# Autodesk Inventor assembly: Final
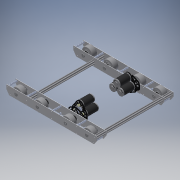
[picture p0: Inventor's stored thumbnail of the model, 180x180]
Saved by Autodesk Inventor 2016 (Build 200138000, 138)
## iProperties
Created: 2017-01-19
Part Number: Final
Document SubType Name: Assembly
Designer: Kyle
Author: Kyle
## Documents named in this file (8)
- C:\Users\Kyle\Documents\FRC1073\FRC1073-CAD\DriveTrain\Final.iam
- C:\Users\Kyle\Documents\FRC1073\FRC1073-CAD\DriveTrain\OutsidePlate.ipt
- C:\Users\Kyle\Documents\FRC1073\FRC1073-CAD\DriveTrain\Individual Parts\Mock 8020 28.25in.ipt
- C:\Users\Kyle\Documents\FRC1073\FRC1073-CAD\DriveTrain\InsidePlate.ipt
- C:\Users\Kyle\Documents\FRC1073\FRC1073-CAD\DriveTrain\Individual Parts\3.625Churro.ipt
- C:\Users\Kyle\Documents\FRC1073\FRC1073-CAD\DriveTrain\Individual Parts\SinglePulley.iam
- C:\Users\Kyle\Documents\FRC1073\FRC1073-CAD\DriveTrain\Individual Parts\DoublePulley.iam
- C:\Users\Kyle\Documents\FRC1073\FRC1073-CAD\DriveTrain\Individual Parts\DoublePulleyGearbox.iam
## Components (32 placed, 7 different names)
1. OutsidePlate:1 — Mate:1, Mate:2, Flush:1, Flush:2, Mate:3, Flush:3, Flush:4, Mate:4, Mate:5, Mate:6, Mate:7, Mate:8, Mate:9, Mate:10, Mate:11, Mate:12, Mate:29, Mate:30, Mate:31, Mate:32, Mate:33, Mate:34, Mate:37, Mate:38
2. Mock 8020 28.25in:1 — Mate:2, Flush:1, Flush:2, Mate:14
3. Mock 8020 28.25in:2 — Mate:1, Mate:3
4. InsidePlate:1 — Flush:3, Flush:4, Mate:13, Mate:42
5. 3.625Churro:1 — Mate:11
6. 3.625Churro:2 — Mate:10, Mate:13
7. 3.625Churro:3 — Mate:12
8. 3.625Churro:4 — Mate:9
9. 3.625Churro:5 — Mate:7
10. 3.625Churro:6 — Mate:8
11. 3.625Churro:7 — Mate:6
12. 3.625Churro:8 — Mate:4
13. 3.625Churro:9 — Mate:5
14. OutsidePlate:2 — Mate:14, Mate:15, Mate:16, Mate:17, Mate:18, Mate:19, Mate:20, Mate:21, Mate:22, Mate:23, Flush:5, Flush:6, Mate:35, Mate:36, Mate:39, Mate:40
15. 3.625Churro:10 — Mate:15
16. 3.625Churro:11 — Mate:16
17. 3.625Churro:12 — Mate:17
18. 3.625Churro:13 — Mate:18
19. 3.625Churro:14 — Mate:19, Mate:24
20. 3.625Churro:15 — Mate:21
21. 3.625Churro:16 — Mate:20
22. 3.625Churro:17 — Mate:23
23. 3.625Churro:18 — Mate:22
24. InsidePlate:2 — Flush:5, Flush:6, Mate:24, Mate:25, Mate:26, Mate:27, Mate:28, Mate:41
25. SinglePulley:1 [sub-assembly] — Mate:31, Mate:32
26. SinglePulley:2 [sub-assembly] — Mate:29, Mate:30
27. SinglePulley:3 [sub-assembly] — Mate:25, Mate:26
28. SinglePulley:4 [sub-assembly] — Mate:27, Mate:28
29. DoublePulley:1 [sub-assembly] — Mate:33, Mate:34
30. DoublePulley:2 [sub-assembly] — Mate:35, Mate:36
31. DoublePulleyGearbox:1 [sub-assembly] — Mate:37, Mate:38, Mate:42
32. DoublePulleyGearbox:2 [sub-assembly] — Mate:39, Mate:40, Mate:41
## Relationships (48: Mate 42, Flush 6)
- Mate:1: OutsidePlate:1 ↔ Mock 8020 28.25in:2
- Mate:2: OutsidePlate:1 ↔ Mock 8020 28.25in:1
- Flush:1 (6.35 mm): OutsidePlate:1 ↔ Mock 8020 28.25in:1
- Flush:2 (6.35 mm): OutsidePlate:1 ↔ Mock 8020 28.25in:1
- Mate:3: OutsidePlate:1 ↔ Mock 8020 28.25in:2
- Flush:3: OutsidePlate:1 ↔ InsidePlate:1
- Flush:4: OutsidePlate:1 ↔ InsidePlate:1
- Mate:4: OutsidePlate:1 ↔ 3.625Churro:8
- Mate:5: OutsidePlate:1 ↔ 3.625Churro:9
- Mate:6: OutsidePlate:1 ↔ 3.625Churro:7
- Mate:7: OutsidePlate:1 ↔ 3.625Churro:5
- Mate:8: OutsidePlate:1 ↔ 3.625Churro:6
- Mate:9: OutsidePlate:1 ↔ 3.625Churro:4
- Mate:10: OutsidePlate:1 ↔ 3.625Churro:2
- Mate:11: OutsidePlate:1 ↔ 3.625Churro:1
- Mate:12: OutsidePlate:1 ↔ 3.625Churro:3
- Mate:13: InsidePlate:1 ↔ 3.625Churro:2
- Mate:14: Mock 8020 28.25in:1 ↔ OutsidePlate:2
- Mate:15: OutsidePlate:2 ↔ 3.625Churro:10
- Mate:16: OutsidePlate:2 ↔ 3.625Churro:11
- Mate:17: OutsidePlate:2 ↔ 3.625Churro:12
- Mate:18: OutsidePlate:2 ↔ 3.625Churro:13
- Mate:19: OutsidePlate:2 ↔ 3.625Churro:14
- Mate:20: OutsidePlate:2 ↔ 3.625Churro:16
- Mate:21: OutsidePlate:2 ↔ 3.625Churro:15
- Mate:22: OutsidePlate:2 ↔ 3.625Churro:18
- Mate:23: OutsidePlate:2 ↔ 3.625Churro:17
- Flush:5: OutsidePlate:2 ↔ InsidePlate:2
- Flush:6: OutsidePlate:2 ↔ InsidePlate:2
- Mate:24: 3.625Churro:14 ↔ InsidePlate:2
- Mate:25: InsidePlate:2 ↔ SinglePulley:3
- Mate:26: InsidePlate:2 ↔ SinglePulley:3
- Mate:27: InsidePlate:2 ↔ SinglePulley:4
- Mate:28: InsidePlate:2 ↔ SinglePulley:4
- Mate:29: OutsidePlate:1 ↔ SinglePulley:2
- Mate:30: OutsidePlate:1 ↔ SinglePulley:2
- Mate:31: OutsidePlate:1 ↔ SinglePulley:1
- Mate:32: OutsidePlate:1 ↔ SinglePulley:1
- Mate:33: OutsidePlate:1 ↔ DoublePulley:1
- Mate:34: OutsidePlate:1 ↔ DoublePulley:1
- Mate:35: OutsidePlate:2 ↔ DoublePulley:2
- Mate:36: OutsidePlate:2 ↔ DoublePulley:2
- Mate:37: OutsidePlate:1 ↔ DoublePulleyGearbox:1
- Mate:38: OutsidePlate:1 ↔ DoublePulleyGearbox:1
- Mate:39: OutsidePlate:2 ↔ DoublePulleyGearbox:2
- Mate:40: OutsidePlate:2 ↔ DoublePulleyGearbox:2
- Mate:41: InsidePlate:2 ↔ DoublePulleyGearbox:2
- Mate:42: InsidePlate:1 ↔ DoublePulleyGearbox:1
